# Autodesk Inventor assembly: DriveChain V3
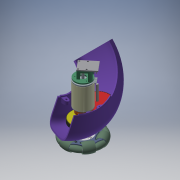
[picture p0: Inventor's stored thumbnail of the model, 180x180]
Saved by Autodesk Inventor 2019.1 (Build 231200000, 200)
## iProperties
Created: 2018-11-14
Part Number: DriveChain V3
Material: Generisch
Document SubType Name: Assembly
Designer: JochenAlt
Author: JochenAlt
## Documents named in this file (7)
- D:\Projects\Ondine\CAD\DriveChain V3.iam
- D:\Projects\Ondine\CAD\DriveChainEnclosure V3.ipt
- D:\Projects\Ondine\CAD\Beltdrive\BeltGear.iam
- D:\Projects\Ondine\CAD\Bearings\W 637_4 X-2Z.iam
- D:\Projects\Ondine\CAD\BeltDriveAxis.ipt
- D:\Projects\Ondine\CAD\OmniWheel.iam
- D:\Projects\Ondine\CAD\BushOmniWheelV3.ipt
## Components (7 placed, 6 different names)
1. DriveChainEnclosure:1 — Passend:1, Passend:2, Passend:3, Passend:4, Passend:12
2. NewBeltGear:1 [sub-assembly] — Passend:5, Passend:6, Passend:9, Passend:10, Passend:11
3. W 637_4 X-2Z:1 [sub-assembly] — Passend:1, Passend:2, Passend:5, Passend:6
4. W 637_4 X-2Z:2 [sub-assembly] — Passend:3, Passend:4, Passend:7, Passend:8
5. HarmonicDrive-Axis:1 — Passend:7, Passend:8, Passend:9
6. OmniWheel:1 [sub-assembly] — Passend:10, Passend:13
7. BushOmniWheel:1 — Passend:11, Passend:12, Passend:13
## Relationships (13: Mate 13)
- Passend:1 [Mate]: DriveChainEnclosure:1 ↔ W 637_4 X-2Z:1
- Passend:2 [Mate]: DriveChainEnclosure:1 ↔ W 637_4 X-2Z:1
- Passend:3 [Mate]: DriveChainEnclosure:1 ↔ W 637_4 X-2Z:2
- Passend:4 [Mate]: DriveChainEnclosure:1 ↔ W 637_4 X-2Z:2
- Passend:5 [Mate]: NewBeltGear:1 ↔ W 637_4 X-2Z:1
- Passend:6 [Mate]: NewBeltGear:1 ↔ W 637_4 X-2Z:1
- Passend:7 [Mate]: W 637_4 X-2Z:2 ↔ HarmonicDrive-Axis:1
- Passend:8 [Mate]: W 637_4 X-2Z:2 ↔ HarmonicDrive-Axis:1
- Passend:9 [Mate]: NewBeltGear:1 ↔ HarmonicDrive-Axis:1
- Passend:10 [Mate]: NewBeltGear:1 ↔ OmniWheel:1
- Passend:11 [Mate]: NewBeltGear:1 ↔ BushOmniWheel:1
- Passend:12 [Mate]: DriveChainEnclosure:1 ↔ BushOmniWheel:1
- Passend:13 [Mate]: OmniWheel:1 ↔ BushOmniWheel:1
